# Autodesk Inventor assembly: frame-and-walls
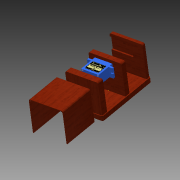
[picture p0: Inventor's stored thumbnail of the model, 180x180]
Saved by Autodesk Inventor 2015 (Build 190159000, 159)
## iProperties
Created: 2014-07-16
Part Number: frame-and-walls
Document SubType Name: Assembly
Designer: pc
Author: pc
## Documents named in this file (8)
- C:\Users\pc\Documents\blinds\inventor\frame-and-walls.iam
- C:\Users\pc\Documents\blinds\inventor\base-frame.ipt
- C:\Users\pc\Documents\blinds\inventor\wall-front.ipt
- C:\Users\pc\Documents\blinds\inventor\wall-middle.ipt
- C:\Users\pc\Documents\blinds\inventor\wall-end.ipt
- C:\Users\pc\Documents\blinds\inventor\back-cover.ipt
- C:\Users\pc\Documents\blinds\inventor\SG90 BODY.ipt
- C:\Users\pc\Documents\blinds\inventor\SG90 ARM.ipt
## Components (7 placed, 6 different names)
1. base-frame:1 — Mate:1, Mate:2, Mate:3, Mate:4, Mate:5, Mate:6, Mate:7, Mate:8, Mate:9, Mate:10
2. Front wall:1 — Mate:1, Mate:2, Mate:3, Mate:12
3. wall-middle:1 — Mate:4, Mate:5, Mate:6, Mate:11, Mate:13, Mate:14, Angle:1
4. wall-end:1 — Mate:7, Mate:8, Mate:9, Mate:10
5. base-frame:2 — Mate:11, Mate:12
6. SG90 BODY:1 — Mate:13, Mate:14, Insert:1
7. SG90 ARM:1 — Insert:1, Angle:1
## Relationships (16: Mate 14, Insert 1, Angle 1)
- Mate:1: base-frame:1 ↔ Front wall:1
- Mate:2: base-frame:1 ↔ Front wall:1
- Mate:3: base-frame:1 ↔ Front wall:1
- Mate:4: base-frame:1 ↔ wall-middle:1
- Mate:5: base-frame:1 ↔ wall-middle:1
- Mate:6: base-frame:1 ↔ wall-middle:1
- Mate:7: base-frame:1 ↔ wall-end:1
- Mate:8: base-frame:1 ↔ wall-end:1
- Mate:9: base-frame:1 ↔ wall-end:1
- Mate:10: base-frame:1 ↔ wall-end:1
- Mate:11: wall-middle:1 ↔ base-frame:2
- Mate:12: Front wall:1 ↔ base-frame:2
- Mate:13: wall-middle:1 ↔ SG90 BODY:1
- Mate:14: wall-middle:1 ↔ SG90 BODY:1
- Insert:1: SG90 BODY:1 ↔ SG90 ARM:1
- Angle:1 (0 deg): wall-middle:1 ↔ SG90 ARM:1
